# Autodesk Inventor assembly: 2v2 LWL Robot
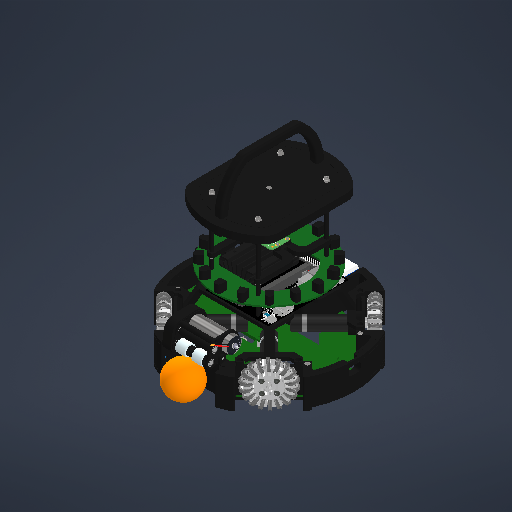
[picture p0: Inventor's stored thumbnail of the model, 512x512]
Saved by Autodesk Inventor 2026.1 (Build 301233020, 233B)
## iProperties
Created: 2025-11-07
Part Number: 2v2 LWL Robot
Document SubType Name: Assembly
Designer: Bahaa
Mass: 992.881 g
Surface Area: 5535.1 cm^2
Volume: 738.435 cm^3
Density: 1.34457 g/cm^3
Author: Bahaa
## Documents named in this file (20)
- C:\Users\Bahaa\Nextcloud2\CAD\25-26\V1\2v2 LWL Robot.iam
- C:\Users\Bahaa\Nextcloud2\CAD\25-26\V1\Bottom Ring.ipt
- C:\Users\Bahaa\Nextcloud2\CAD\25-26\V1\Boards\Line Board.ipt
- C:\Users\Bahaa\Nextcloud2\CAD\25-26\V1\Motor Assembly.iam
- C:\Users\Bahaa\Nextcloud2\CAD\25-26\V1\Side Wall.ipt
- C:\Users\Bahaa\Nextcloud2\CAD\25-26\V1\Top Ring.ipt
- C:\Users\Bahaa\Nextcloud2\CAD\25-26\V1\Solenoid.iam
- C:\Users\Bahaa\Nextcloud2\CAD\25-26\V1\Ball.ipt
- C:\Users\Bahaa\Nextcloud2\CAD\25-26\V1\Boards\Solenoid Board.ipt
- C:\Users\Bahaa\Nextcloud2\CAD\25-26\V1\Boards\Main Board w. Parts.iam
- C:\Users\Bahaa\Nextcloud2\CAD\25-26\V1\Central Assembly.iam
- C:\Users\Bahaa\Nextcloud2\CAD\25-26\V1\Dribbler\Dribbler.iam
- C:\Users\Bahaa\Nextcloud2\CAD\25-26\V1\Side Wall Teensy.ipt
- C:\Users\Bahaa\Nextcloud2\CAD\25-26\V1\Battery Cover.ipt
- C:\Users\Bahaa\Documents\Inventor\Content Center Files\R2026\en-US\DIN 912\DIN 912 - M3 x 0,5 x 20 x 18,75.ipt
- C:\Users\Bahaa\Documents\Inventor\Content Center Files\R2026\en-US\DIN 912\DIN 912 - M3 x 0,5 x 5 x 3,75.ipt
- C:\Users\Bahaa\Nextcloud2\CAD\25-26\V1\Parts\WP3DP3BT angled.ipt
- C:\Users\Bahaa\Nextcloud2\CAD\25-26\V1\Parts\LED angled.ipt
- C:\Users\Bahaa\Nextcloud2\CAD\25-26\V1\Parts\SLS X-CUBE 1250mAh 3S1P 11,1V 60.ipt
- C:\Users\Bahaa\Nextcloud2\CAD\25-26\V1\Ground Cover.ipt
## Components (32 placed, 19 different names)
1. Ground Cover:1 — Mate:153, Mate:154, Mate:155, Mate:156, Mate:157, Mate:158
2. Bottom Ring:1 — Flush:1, Flush:2, Mate:1, Mate:2, Mate:7, Mate:8, Mate:9, Mate:10, Mate:23, Mate:108, Mate:122, Mate:126, Mate:127, Mate:128, Mate:129, Mate:131, Insert:10, Insert:11, Insert:12, Insert:13, Insert:14, Mate:136, Mate:137, Angle:5, Mate:138, Mate:139, Angle:6, Mate:151, Mate:153
3. Line Board:1 — Mate:2, Mate:77, Mate:78, Mate:90, Mate:108, Mate:109, Mate:150, Mate:154, Mate:155, Mate:156, Mate:157, Mate:158
4. Side Wall:1 — Mate:10, Mate:125, Mate:126, Mate:127
5. Top Ring:1 — Flush:5, Flush:6, Mate:31, Mate:32, Mate:123, Mate:124, Mate:125, Mate:132, Insert:1, Insert:3, Insert:4, Insert:5, Insert:8, Insert:9, Mate:135, Mate:143, Mate:144, Mate:145, Mate:149, Mate:152, Mate:159, Mate:160, Mate:161
6. Solenoid:2 [sub-assembly] — Flush:5, Flush:6, Mate:22, Mate:135
7. Ball:1 — Mate:22, Mate:23, Mate:24
8. Solenoid Board:1 — Mate:149
9. Main Board w. Parts:1 [sub-assembly] — Mate:77, Mate:78, Mate:90
10. Side Wall Teensy:1 — Mate:122, Mate:123, Mate:124
11. Battery Cover:1 — Mate:128, Mate:129, Mate:130, Mate:132
12. WP3DP3BT angled:1 — Mate:136, Mate:137, Angle:5
13. LED angled:1 — Mate:138, Mate:139, Angle:6
14. Central Assembly:1 [sub-assembly] — Mate:159, Mate:160, Mate:161
15. Dribbler:1 [sub-assembly] — Mate:143, Mate:144, Mate:145
16. SLS X-CUBE 1250mAh 3S1P 11,1V 60:1 — Mate:150, Mate:151, Mate:152
17. DIN 912 - replaced by DIN EN ISO 4762 M3 x 20:1 — Mate:130, Mate:131
18. DIN 912 - replaced by DIN EN ISO 4762 M3 x 5:1 — Insert:1
19. DIN 912 - replaced by DIN EN ISO 4762 M3 x 5:3 — Insert:3
20. DIN 912 - replaced by DIN EN ISO 4762 M3 x 5:4 — Insert:4
21. DIN 912 - replaced by DIN EN ISO 4762 M3 x 5:5 — Insert:5
22. DIN 912 - replaced by DIN EN ISO 4762 M3 x 5:8 — Insert:8
23. DIN 912 - replaced by DIN EN ISO 4762 M3 x 5:9 — Insert:9
24. DIN 912 - replaced by DIN EN ISO 4762 M3 x 5:10 — Insert:10
25. DIN 912 - replaced by DIN EN ISO 4762 M3 x 5:11 — Insert:11
26. DIN 912 - replaced by DIN EN ISO 4762 M3 x 5:12 — Insert:12
27. DIN 912 - replaced by DIN EN ISO 4762 M3 x 5:13 — Insert:13
28. DIN 912 - replaced by DIN EN ISO 4762 M3 x 5:14 — Insert:14
29. Motor Assembly:1 [sub-assembly] — Mate:7, Mate:8, Mate:9
30. Motor Assembly:2 [sub-assembly] — Flush:7
31. Motor Assembly:3 [sub-assembly] — Mate:32, Mate:109
32. Motor Assembly:4 [sub-assembly] — Mate:31
## Component patterns: Motor Assemblies (4 elements)
## Relationships (66: Mate 48, Insert 11, Flush 5, Angle 2)
- Flush:1: Bottom Ring:1
- Flush:2: Bottom Ring:1
- Mate:1: Bottom Ring:1
- Mate:2: Bottom Ring:1 ↔ Line Board:1
- Mate:7: Bottom Ring:1 ↔ Motor Assembly:1
- Mate:8: Bottom Ring:1 ↔ Motor Assembly:1
- Mate:9: Bottom Ring:1 ↔ Motor Assembly:1
- Mate:10: Bottom Ring:1 ↔ Side Wall:1
- Flush:5: Top Ring:1 ↔ Solenoid:2
- Flush:6: Top Ring:1 ↔ Solenoid:2
- Mate:22 (21 mm): Solenoid:2 ↔ Ball:1
- Mate:23 (32.5 mm): Bottom Ring:1 ↔ Ball:1
- Flush:7 (11.3398 mm): Motor Assembly:2
- Mate:24 (-21 mm): Ball:1
- Mate:31: Top Ring:1 ↔ Motor Assembly:4
- Mate:32: Top Ring:1 ↔ Motor Assembly:3
- Mate:77: Line Board:1 ↔ Main Board w. Parts:1
- Mate:78: Line Board:1 ↔ Main Board w. Parts:1
- Mate:90: Line Board:1 ↔ Main Board w. Parts:1
- Mate:108: Bottom Ring:1 ↔ Line Board:1
- Mate:109: Line Board:1 ↔ Motor Assembly:3
- Mate:122: Bottom Ring:1 ↔ Side Wall Teensy:1
- Mate:123: Top Ring:1 ↔ Side Wall Teensy:1
- Mate:124: Top Ring:1 ↔ Side Wall Teensy:1
- Mate:125: Side Wall:1 ↔ Top Ring:1
- Mate:126: Bottom Ring:1 ↔ Side Wall:1
- Mate:127: Bottom Ring:1 ↔ Side Wall:1
- Mate:128: Bottom Ring:1 ↔ Battery Cover:1
- Mate:129: Bottom Ring:1 ↔ Battery Cover:1
- Mate:130: Battery Cover:1 ↔ DIN 912 - replaced by DIN EN ISO 4762 M3 x 20:1
- Mate:131: Bottom Ring:1 ↔ DIN 912 - replaced by DIN EN ISO 4762 M3 x 20:1
- Mate:132: Top Ring:1 ↔ Battery Cover:1
- Insert:1: Top Ring:1 ↔ DIN 912 - replaced by DIN EN ISO 4762 M3 x 5:1
- Insert:3: Top Ring:1 ↔ DIN 912 - replaced by DIN EN ISO 4762 M3 x 5:3
- Insert:4: Top Ring:1 ↔ DIN 912 - replaced by DIN EN ISO 4762 M3 x 5:4
- Insert:5: Top Ring:1 ↔ DIN 912 - replaced by DIN EN ISO 4762 M3 x 5:5
- Insert:8: Top Ring:1 ↔ DIN 912 - replaced by DIN EN ISO 4762 M3 x 5:8
- Insert:9: Top Ring:1 ↔ DIN 912 - replaced by DIN EN ISO 4762 M3 x 5:9
- Insert:10: Bottom Ring:1 ↔ DIN 912 - replaced by DIN EN ISO 4762 M3 x 5:10
- Insert:11: Bottom Ring:1 ↔ DIN 912 - replaced by DIN EN ISO 4762 M3 x 5:11
- Insert:12: Bottom Ring:1 ↔ DIN 912 - replaced by DIN EN ISO 4762 M3 x 5:12
- Insert:13: Bottom Ring:1 ↔ DIN 912 - replaced by DIN EN ISO 4762 M3 x 5:13
- Insert:14: Bottom Ring:1 ↔ DIN 912 - replaced by DIN EN ISO 4762 M3 x 5:14
- Mate:135: Top Ring:1 ↔ Solenoid:2
- Mate:136 (3 mm): Bottom Ring:1 ↔ WP3DP3BT angled:1
- Mate:137: Bottom Ring:1 ↔ WP3DP3BT angled:1
- Angle:5 (180 deg): Bottom Ring:1 ↔ WP3DP3BT angled:1
- Mate:138 (3 mm): Bottom Ring:1 ↔ LED angled:1
- Mate:139: Bottom Ring:1 ↔ LED angled:1
- Angle:6 (0 deg): Bottom Ring:1 ↔ LED angled:1
- Mate:143: Top Ring:1 ↔ Dribbler:1
- Mate:144: Top Ring:1 ↔ Dribbler:1
- Mate:145: Top Ring:1 ↔ Dribbler:1
- Mate:149: Top Ring:1 ↔ Solenoid Board:1
- Mate:150: Line Board:1 ↔ SLS X-CUBE 1250mAh 3S1P 11,1V 60:1
- Mate:151 (0.25 mm): Bottom Ring:1 ↔ SLS X-CUBE 1250mAh 3S1P 11,1V 60:1
- Mate:152: Top Ring:1 ↔ SLS X-CUBE 1250mAh 3S1P 11,1V 60:1
- Mate:153: Ground Cover:1 ↔ Bottom Ring:1
- Mate:154: Ground Cover:1 ↔ Line Board:1
- Mate:155: Ground Cover:1 ↔ Line Board:1
- Mate:156: Ground Cover:1 ↔ Line Board:1
- Mate:157: Ground Cover:1 ↔ Line Board:1
- Mate:158: Ground Cover:1 ↔ Line Board:1
- Mate:159: Top Ring:1 ↔ Central Assembly:1
- Mate:160: Top Ring:1 ↔ Central Assembly:1
- Mate:161: Top Ring:1 ↔ Central Assembly:1
